# Autodesk Inventor assembly: circle sheet assemble
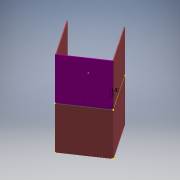
[picture p0: Inventor's stored thumbnail of the model, 180x180]
Saved by Autodesk Inventor 2019 (Build 230136000, 136)
## iProperties
Created: 2020-03-05
Part Number: circle sheet assemble
Document SubType Name: Assembly
Designer: Hp
Author: Hp
## Documents named in this file (11)
- C:\Users\Hp\Desktop\expooooooooooooooooo\epolaration model\circle sheet assemble.iam
- C:\Users\Hp\Desktop\expooooooooooooooooo\epolaration model\circle sheet.ipt
- C:\Users\Hp\Desktop\expooooooooooooooooo\epolaration model\Part6.ipt
- C:\Users\Hp\Desktop\expooooooooooooooooo\epolaration model\dc motor.ipt
- C:\Users\Hp\Desktop\expooooooooooooooooo\epolaration model\steeper.ipt
- C:\Users\Hp\Desktop\expooooooooooooooooo\epolaration model\circle.ipt
- C:\Users\Hp\Desktop\expooooooooooooooooo\epolaration model\arrow.ipt
- C:\Users\Hp\Desktop\expooooooooooooooooo\epolaration model\colour.ipt
- C:\Users\Hp\Desktop\expooooooooooooooooo\epolaration model\side walls.ipt
- C:\Users\Hp\Desktop\expooooooooooooooooo\epolaration model\key.ipt
- C:\Users\Hp\Desktop\expooooooooooooooooo\epolaration model\upper shheet.ipt
## Components (27 placed, 10 different names)
1. circle sheet:1 — Rotational:1, Rotational:2, Rotational:3, Rigid:3, Rigid:4, Rigid:5, Rotational:9, Rotational:10, Rigid:7
2. Part6:1 — Rotational:2, Rotational:4, Rotational:7
3. Part6:2 — Rotational:3, Rotational:6
4. Part6:3 — Rotational:1, Rigid:1
5. Part6:4 — Rotational:4, Rotational:8
6. dc motor:1 — Rigid:1
7. circle:1 — Rotational:6
8. arrow:1 — Rotational:8, Rigid:2
9. steeper:1 — Rotational:7
10. colour:1 — Rigid:2
11. side walls:1 — Rigid:3
12. side walls:2 — Rigid:5, Rigid:6
13. side walls:3 — Rigid:4
14. side walls:4 — Rigid:6
15. Part6:5 — Rotational:9, Rotational:11
16. Part6:6 — Rotational:10
17. key:1 — Rotational:11
18. upper shheet:1 — Rigid:7, Rigid:8, Rigid:9, Rotational:12, Rotational:13, Rotational:14, Rotational:15, Rotational:16, Rotational:17, Rotational:18
19. side walls:6 — Rigid:8
20. side walls:7 — Rigid:9
21. Part6:7 — Rotational:14
22. Part6:8 — Rotational:15
23. Part6:9 — Rotational:12
24. Part6:10 — Rotational:13
25. Part6:11 — Rotational:16
26. Part6:12 — Rotational:17
27. Part6:13 — Rotational:18
## Relationships (26: RevoluteJoint 17, WeldJoint 9)
- Rotational:1 [RevoluteJoint]: circle sheet:1 ↔ Part6:3
- Rotational:2 [RevoluteJoint]: circle sheet:1 ↔ Part6:1
- Rotational:3 [RevoluteJoint]: circle sheet:1 ↔ Part6:2
- Rotational:4 [RevoluteJoint]: Part6:1 ↔ Part6:4
- Rigid:1 [WeldJoint]: Part6:3 ↔ dc motor:1
- Rotational:6 [RevoluteJoint]: Part6:2 ↔ circle:1
- Rotational:7 [RevoluteJoint] (5 mm): Part6:1 ↔ steeper:1
- Rotational:8 [RevoluteJoint]: Part6:4 ↔ arrow:1
- Rigid:2 [WeldJoint]: arrow:1 ↔ colour:1
- Rigid:3 [WeldJoint]: circle sheet:1 ↔ side walls:1
- Rigid:4 [WeldJoint]: circle sheet:1 ↔ side walls:3
- Rigid:5 [WeldJoint]: circle sheet:1 ↔ side walls:2
- Rigid:6 [WeldJoint]: side walls:2 ↔ side walls:4
- Rotational:9 [RevoluteJoint]: circle sheet:1 ↔ Part6:5
- Rotational:10 [RevoluteJoint]: circle sheet:1 ↔ Part6:6
- Rotational:11 [RevoluteJoint]: Part6:5 ↔ key:1
- Rigid:7 [WeldJoint]: circle sheet:1 ↔ upper shheet:1
- Rigid:8 [WeldJoint]: upper shheet:1 ↔ side walls:6
- Rigid:9 [WeldJoint]: upper shheet:1 ↔ side walls:7
- Rotational:12 [RevoluteJoint]: upper shheet:1 ↔ Part6:9
- Rotational:13 [RevoluteJoint]: upper shheet:1 ↔ Part6:10
- Rotational:14 [RevoluteJoint]: upper shheet:1 ↔ Part6:7
- Rotational:15 [RevoluteJoint]: upper shheet:1 ↔ Part6:8
- Rotational:16 [RevoluteJoint]: upper shheet:1 ↔ Part6:11
- Rotational:17 [RevoluteJoint]: upper shheet:1 ↔ Part6:12
- Rotational:18 [RevoluteJoint]: upper shheet:1 ↔ Part6:13
